# Autodesk Inventor assembly: Wind Tunnel Settling Chamber As-Built
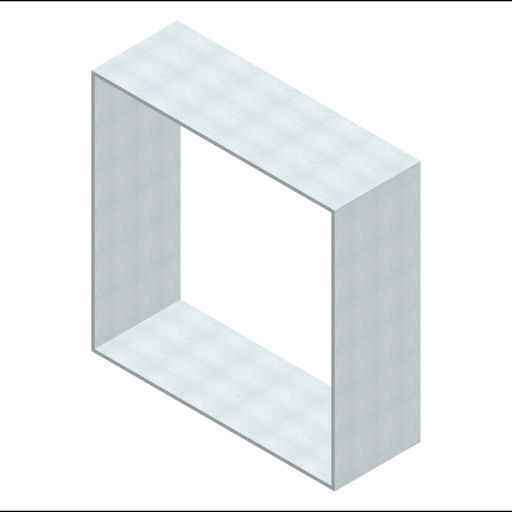
[picture p0: Inventor's stored thumbnail of the model, 512x512]
Saved by Autodesk Inventor 2023 (Build 270158000, 158)
## iProperties
Created: 2023-01-19
Part Number: Wind Tunnel Settling Chamber As-Built
Document SubType Name: Assembly
Designer: kamer
Author: kamer
## Documents named in this file (3)
- X:\Storage\Documents\ME 306 Heat Transfer Project Files\CAD\Wind Tunnel Settling Chamber As-Built.iam
- X:\Storage\Documents\ME 306 Heat Transfer Project Files\CAD\Wind Tunnel Settling Chamber Top+Bottom As-Built.ipt
- X:\Storage\Documents\ME 306 Heat Transfer Project Files\CAD\Wind Tunnel Settling Chamber Side As-Built.ipt
## Components (4 placed, 2 different names)
1. Wind Tunnel Settling Chamber Top+Bottom As-Built:1 — Flush:1, Flush:2, Mate:1, Flush:3, Flush:4, Mate:2, Flush:5, Mate:3, Flush:6
2. Wind Tunnel Settling Chamber Top+Bottom As-Built:2 — Flush:1, Flush:2, Mate:1
3. Wind Tunnel Settling Chamber Side As-Built:1 — Flush:5, Mate:3, Flush:6
4. Wind Tunnel Settling Chamber Side As-Built:2 — Flush:3, Flush:4, Mate:2
## Relationships (9: Flush 6, Mate 3)
- Flush:1: Wind Tunnel Settling Chamber Top+Bottom As-Built:1 ↔ Wind Tunnel Settling Chamber Top+Bottom As-Built:2
- Flush:2: Wind Tunnel Settling Chamber Top+Bottom As-Built:1 ↔ Wind Tunnel Settling Chamber Top+Bottom As-Built:2
- Mate:1 (838.2 mm): Wind Tunnel Settling Chamber Top+Bottom As-Built:1 ↔ Wind Tunnel Settling Chamber Top+Bottom As-Built:2
- Flush:3: Wind Tunnel Settling Chamber Top+Bottom As-Built:1 ↔ Wind Tunnel Settling Chamber Side As-Built:2
- Flush:4: Wind Tunnel Settling Chamber Top+Bottom As-Built:1 ↔ Wind Tunnel Settling Chamber Side As-Built:2
- Mate:2: Wind Tunnel Settling Chamber Top+Bottom As-Built:1 ↔ Wind Tunnel Settling Chamber Side As-Built:2
- Flush:5: Wind Tunnel Settling Chamber Top+Bottom As-Built:1 ↔ Wind Tunnel Settling Chamber Side As-Built:1
- Mate:3: Wind Tunnel Settling Chamber Top+Bottom As-Built:1 ↔ Wind Tunnel Settling Chamber Side As-Built:1
- Flush:6: Wind Tunnel Settling Chamber Top+Bottom As-Built:1 ↔ Wind Tunnel Settling Chamber Side As-Built:1
